# Autodesk Inventor assembly: Leg
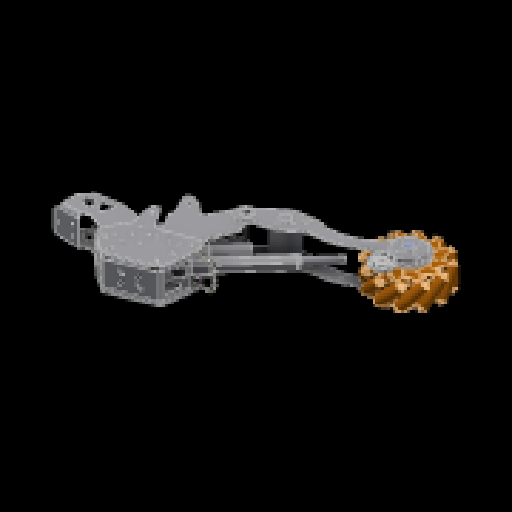
[picture p0: Inventor's stored thumbnail of the model, 512x512]
Saved by Autodesk Inventor 2025.2 (Build 292293000, 293)
## iProperties
Created: 2020-05-17
Part Number: Leg
Document SubType Name: Assembly
Designer: valer
_SolveAssemblyDoc: Frame Generator Solve Assembly
_Version: 15.0.0
Author: valer
## Documents named in this file (25)
- C:\Users\valer\Desktop\str1ker\cad\Leg.iam
- C:\Users\valer\Desktop\str1ker\cad\LegThigh.ipt
- C:\Users\valer\Desktop\str1ker\cad\LegShin.ipt
- C:\Users\valer\Desktop\str1ker\cad\LegHipSide.ipt
- C:\Users\valer\Desktop\str1ker\cad\LegHip.ipt
- C:\Users\valer\Desktop\str1ker\cad\LegHipFront.ipt
- C:\Users\valer\Desktop\str1ker\cad\external\2796N15_Omni-Directional Wheel.ipt
- C:\Users\valer\Desktop\str1ker\cad\external\MY6812-12VDC-120W-Motor.ipt
- C:\Users\valer\Desktop\str1ker\cad\external\SprocketMDEOOSKY-25H-47T.ipt
- C:\Users\valer\Desktop\str1ker\cad\LegHub.ipt
- C:\Users\valer\Desktop\str1ker\cad\external\6656K234_Ultra-Thin Ball Bearing.ipt
- C:\Users\valer\Desktop\str1ker\cad\LegInsideConnector.ipt
- C:\Users\valer\Desktop\str1ker\cad\LegHandleDesign.ipt
- C:\Users\valer\Desktop\str1ker\cad\external\Hub8mm.ipt
- C:\Users\valer\Desktop\str1ker\cad\LegFrame\LegFrame.iam
- C:\Users\valer\Desktop\str1ker\cad\external\WheelEncoder\am-4027 CIM_Coder_256_Encoder.iam
- C:\Users\valer\Desktop\str1ker\cad\external\WheelEncoder\am-4027 CIM_Coder_256_Magnet.iam
- C:\Users\valer\Desktop\str1ker\cad\CimCoderMount.ipt
- C:\Users\valer\Desktop\str1ker\cad\external\LegActuator\FA-PO-XXX-12-4-Body.ipt
- C:\Users\valer\Desktop\str1ker\cad\external\LegActuator\FA-PO-XXX-12-4-Shaft.ipt
- C:\Users\valer\Desktop\str1ker\cad\LegEncoderHub.ipt
- C:\Users\valer\Desktop\str1ker\cad\external\LegChainRollerGuide.ipt
- C:\Users\valer\Desktop\str1ker\cad\LegKneeShaft.ipt
- C:\Users\valer\Desktop\str1ker\cad\external\91273A406_Same-Size Thread 18-8 Stainless Steel Shoulder Screw.ipt
- C:\Users\valer\Desktop\str1ker\cad\external\91290A185_Black-Oxide Alloy Steel Socket Head Screw.ipt
## Components (37 placed, 24 different names)
1. LegThigh:1 — Flush:1, Mate:1, Mate:4, Mate:163, Mate:250
2. LegHipSide:1 — Flush:1, Mate:1, Mate:4, Flush:140, Flush:141, Mate:152, Mate:153, Mate:154, Angle:2, Mate:161, Mate:168, Mate:171, Mate:180, Mate:222
3. LegThigh:2 — Mate:133, Mate:139, Mate:145, Mate:146, Mate:249, Mate:267
4. LegHipSide:2 — Mate:145, Mate:146, Flush:140, Flush:141, Mate:156
5. MY6812-12VDC-120W-Motor:1 — Mate:77, Mate:80, Mate:89, Mate:93, Flush:4, Flush:5, Mate:132, Mate:182
6. LegShin:3 — Mate:77, Mate:80, Mate:163, Mate:175, Mate:182, Mate:184, Mate:217, Mate:247, Mate:248, Mate:251, Mate:254
7. LegShin:4 — Mate:89, Mate:132, Mate:133, Mate:139, Mate:177, Mate:216, Mate:217, Mate:220, Mate:223, Flush:148, Mate:240, Mate:241, Mate:243, Mate:244
8. SprocketMDEOOSKY-25H-47T:1 — Flush:4, Mate:96, Mate:110, Flush:5, Mate:181, Mate:184
9. LegHub:1 — Mate:97, Mate:108, Mate:109, Mate:110, Mate:181, Mate:255, Mate:256, Mate:257, Mate:258, Mate:259, Mate:260, Mate:261, Mate:262, Mate:263, Mate:264, Mate:265, Mate:266
10. 2796N15_Omni-Directional Wheel:1 — Mate:96, Mate:97, Mate:103, Mate:104, Mate:108, Mate:109, Mate:231, Mate:235
11. 6656K234_Ultra-Thin Ball Bearing:1 — Mate:223, Flush:148, Mate:227
12. 6656K234_Ultra-Thin Ball Bearing:2 — Mate:103, Mate:104
13. LegHandleDesign:1 — Flush:143, Mate:170, Mate:171
14. LegHip:1 — Mate:152, Mate:153, Mate:154, Mate:155, Mate:157, Mate:164, Flush:142, Mate:178
15. LegInsideConnector:5 — Mate:155, Mate:156, Mate:157, Mate:162, Mate:179, Mate:267
16. LegHipFront:1 — Angle:2, Mate:161, Mate:162, Mate:165
17. Hub8mm:1 — Mate:175, Mate:246, Mate:247, Mate:248
18. Hub8mm:2 — Mate:177, Mate:216
19. LegInsideConnector:6 — Mate:178, Mate:179, Mate:180
20. LegFrame:1 [sub-assembly]
21. am-4027 CIM_Coder_256_Encoder:1 [sub-assembly] — Mate:237, Mate:238, Mate:268
22. CimCoderMount:1 — Mate:238, Mate:240, Mate:241
23. FA-PO-XXX-12-4-Body:1 — Flush:147, Mate:219, Mate:222
24. FA-PO-XXX-12-4-Shaft:1 — Mate:219, Mate:220
25. am-4027 CIM_Coder_256_Magnet:1 [sub-assembly] — Mate:232, Mate:236, Mate:237, Mate:242, Mate:268
26. LegEncoderHub:1 — Mate:227, Mate:231, Mate:232, Mate:233, Angle:150, Mate:234, Mate:235
27. Hub8mm:3 — Mate:233, Angle:150, Mate:234, Mate:236
28. CimCoderMount:2 — Mate:242, Mate:243, Mate:244
29. LegChainRollerGuide:1 — Mate:252, Mate:253
30. LegKneeShaft:1 — Mate:246, Mate:249, Mate:250
31. 91273A406_Same-Size Thread 18-8 Stainless Steel Shoulder Screw:1 — Mate:251, Mate:252, Mate:253, Mate:254
32. 91290A185_Black-Oxide Alloy Steel Socket Head Screw:1 — Mate:255, Mate:256
33. 91290A185_Black-Oxide Alloy Steel Socket Head Screw:2 — Mate:257, Mate:258
34. 91290A185_Black-Oxide Alloy Steel Socket Head Screw:3 — Mate:259, Mate:260
35. 91290A185_Black-Oxide Alloy Steel Socket Head Screw:4 — Mate:261, Mate:262
36. 91290A185_Black-Oxide Alloy Steel Socket Head Screw:5 — Mate:263, Mate:264
37. 91290A185_Black-Oxide Alloy Steel Socket Head Screw:6 — Mate:265, Mate:266
## Relationships (95: Mate 83, Flush 9, Angle 3)
- Flush:1 (-5.08 mm): LegThigh:1 ↔ LegHipSide:1
- Mate:1: LegThigh:1 ↔ LegHipSide:1
- Mate:4: LegThigh:1 ↔ LegHipSide:1
- Mate:77: MY6812-12VDC-120W-Motor:1 ↔ LegShin:3
- Mate:80: MY6812-12VDC-120W-Motor:1 ↔ LegShin:3
- Mate:89: MY6812-12VDC-120W-Motor:1 ↔ LegShin:4
- Mate:93: MY6812-12VDC-120W-Motor:1
- Flush:4: MY6812-12VDC-120W-Motor:1 ↔ SprocketMDEOOSKY-25H-47T:1
- Mate:96: SprocketMDEOOSKY-25H-47T:1 ↔ 2796N15_Omni-Directional Wheel:1
- Mate:97: LegHub:1 ↔ 2796N15_Omni-Directional Wheel:1
- Mate:103: 2796N15_Omni-Directional Wheel:1 ↔ 6656K234_Ultra-Thin Ball Bearing:2
- Mate:104: 2796N15_Omni-Directional Wheel:1 ↔ 6656K234_Ultra-Thin Ball Bearing:2
- Mate:108: LegHub:1 ↔ 2796N15_Omni-Directional Wheel:1
- Mate:109: LegHub:1 ↔ 2796N15_Omni-Directional Wheel:1
- Mate:110: SprocketMDEOOSKY-25H-47T:1 ↔ LegHub:1
- Flush:5: MY6812-12VDC-120W-Motor:1 ↔ SprocketMDEOOSKY-25H-47T:1
- Mate:132: MY6812-12VDC-120W-Motor:1 ↔ LegShin:4
- Mate:133: LegThigh:2 ↔ LegShin:4
- Mate:139: LegThigh:2 ↔ LegShin:4
- Mate:145: LegThigh:2 ↔ LegHipSide:2
- Mate:146: LegThigh:2 ↔ LegHipSide:2
- Flush:140: LegHipSide:1 ↔ LegHipSide:2
- Flush:141: LegHipSide:1 ↔ LegHipSide:2
- Mate:152: LegHipSide:1 ↔ LegHip:1
- Mate:153: LegHipSide:1 ↔ LegHip:1
- Mate:154: LegHipSide:1 ↔ LegHip:1
- Mate:155: LegHip:1 ↔ LegInsideConnector:5
- Mate:156: LegHipSide:2 ↔ LegInsideConnector:5
- Mate:157: LegHip:1 ↔ LegInsideConnector:5
- Angle:2 (0 deg): LegHipSide:1 ↔ LegHipFront:1
- Mate:161: LegHipSide:1 ↔ LegHipFront:1
- Mate:162: LegInsideConnector:5 ↔ LegHipFront:1
- Mate:163: LegThigh:1 ↔ LegShin:3
- Mate:164: LegHip:1
- Mate:165: LegHipFront:1
- Flush:142: LegHip:1
- Mate:168: LegHipSide:1
- Angle:3 (0 deg)
- Flush:143: LegHandleDesign:1
- Mate:170: LegHandleDesign:1
- Mate:171: LegHipSide:1 ↔ LegHandleDesign:1
- Mate:175: LegShin:3 ↔ Hub8mm:1
- Mate:177: LegShin:4 ↔ Hub8mm:2
- Mate:178: LegHip:1 ↔ LegInsideConnector:6
- Mate:179: LegInsideConnector:5 ↔ LegInsideConnector:6
- Mate:180: LegHipSide:1 ↔ LegInsideConnector:6
- Mate:181: SprocketMDEOOSKY-25H-47T:1 ↔ LegHub:1
- Mate:182: MY6812-12VDC-120W-Motor:1 ↔ LegShin:3
- Mate:184: LegShin:3 ↔ SprocketMDEOOSKY-25H-47T:1
- Mate:216: LegShin:4 ↔ Hub8mm:2
- Mate:217: LegShin:3 ↔ LegShin:4
- Flush:147: FA-PO-XXX-12-4-Body:1
- Mate:219: FA-PO-XXX-12-4-Body:1 ↔ FA-PO-XXX-12-4-Shaft:1
- Mate:220: LegShin:4 ↔ FA-PO-XXX-12-4-Shaft:1
- Mate:222: LegHipSide:1 ↔ FA-PO-XXX-12-4-Body:1
- Mate:223: LegShin:4 ↔ 6656K234_Ultra-Thin Ball Bearing:1
- Flush:148: LegShin:4 ↔ 6656K234_Ultra-Thin Ball Bearing:1
- Mate:227: 6656K234_Ultra-Thin Ball Bearing:1 ↔ LegEncoderHub:1
- Mate:231: 2796N15_Omni-Directional Wheel:1 ↔ LegEncoderHub:1
- Mate:232: am-4027 CIM_Coder_256_Magnet:1 ↔ LegEncoderHub:1
- Mate:233: LegEncoderHub:1 ↔ Hub8mm:3
- Angle:150 (0 deg): LegEncoderHub:1 ↔ Hub8mm:3
- Mate:234: LegEncoderHub:1 ↔ Hub8mm:3
- Mate:235: 2796N15_Omni-Directional Wheel:1 ↔ LegEncoderHub:1
- Mate:236: am-4027 CIM_Coder_256_Magnet:1 ↔ Hub8mm:3
- Mate:237: am-4027 CIM_Coder_256_Encoder:1 ↔ am-4027 CIM_Coder_256_Magnet:1
- Mate:238: am-4027 CIM_Coder_256_Encoder:1 ↔ CimCoderMount:1
- Mate:240: LegShin:4 ↔ CimCoderMount:1
- Mate:241: LegShin:4 ↔ CimCoderMount:1
- Mate:242: am-4027 CIM_Coder_256_Magnet:1 ↔ CimCoderMount:2
- Mate:243: LegShin:4 ↔ CimCoderMount:2
- Mate:244: LegShin:4 ↔ CimCoderMount:2
- Mate:246: Hub8mm:1 ↔ LegKneeShaft:1
- Mate:247: LegShin:3 ↔ Hub8mm:1
- Mate:248: LegShin:3 ↔ Hub8mm:1
- Mate:249: LegThigh:2 ↔ LegKneeShaft:1
- Mate:250: LegThigh:1 ↔ LegKneeShaft:1
- Mate:251: LegShin:3 ↔ 91273A406_Same-Size Thread 18-8 Stainless Steel Shoulder Screw:1
- Mate:252: LegChainRollerGuide:1 ↔ 91273A406_Same-Size Thread 18-8 Stainless Steel Shoulder Screw:1
- Mate:253: LegChainRollerGuide:1 ↔ 91273A406_Same-Size Thread 18-8 Stainless Steel Shoulder Screw:1
- Mate:254: LegShin:3 ↔ 91273A406_Same-Size Thread 18-8 Stainless Steel Shoulder Screw:1
- Mate:255: LegHub:1 ↔ 91290A185_Black-Oxide Alloy Steel Socket Head Screw:1
- Mate:256: LegHub:1 ↔ 91290A185_Black-Oxide Alloy Steel Socket Head Screw:1
- Mate:257: LegHub:1 ↔ 91290A185_Black-Oxide Alloy Steel Socket Head Screw:2
- Mate:258: LegHub:1 ↔ 91290A185_Black-Oxide Alloy Steel Socket Head Screw:2
- Mate:259: LegHub:1 ↔ 91290A185_Black-Oxide Alloy Steel Socket Head Screw:3
- Mate:260: LegHub:1 ↔ 91290A185_Black-Oxide Alloy Steel Socket Head Screw:3
- Mate:261: LegHub:1 ↔ 91290A185_Black-Oxide Alloy Steel Socket Head Screw:4
- Mate:262: LegHub:1 ↔ 91290A185_Black-Oxide Alloy Steel Socket Head Screw:4
- Mate:263: LegHub:1 ↔ 91290A185_Black-Oxide Alloy Steel Socket Head Screw:5
- Mate:264: LegHub:1 ↔ 91290A185_Black-Oxide Alloy Steel Socket Head Screw:5
- Mate:265: LegHub:1 ↔ 91290A185_Black-Oxide Alloy Steel Socket Head Screw:6
- Mate:266: LegHub:1 ↔ 91290A185_Black-Oxide Alloy Steel Socket Head Screw:6
- Mate:267: LegThigh:2 ↔ LegInsideConnector:5
- Mate:268: am-4027 CIM_Coder_256_Encoder:1 ↔ am-4027 CIM_Coder_256_Magnet:1
